# Autodesk Inventor assembly: ZespolDuzegoKola
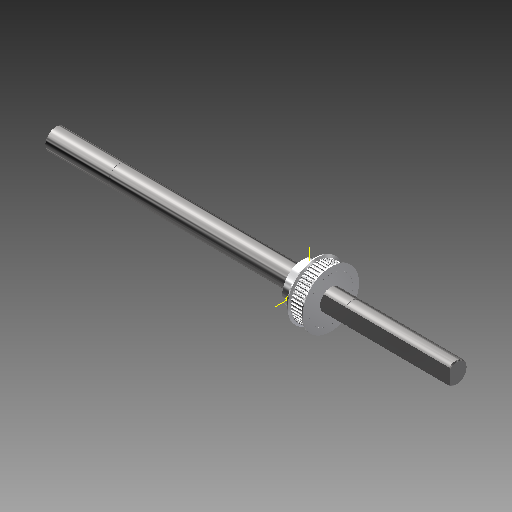
[picture p0: Inventor's stored thumbnail of the model, 512x512]
Saved by Autodesk Inventor 2019 (Build 230136000, 136)
## iProperties
Created: 2020-05-23
Part Number: ZespolDuzegoKola
Document SubType Name: Assembly
Designer: estee
Author: estee
## Documents named in this file (4)
- C:\Users\estee\OneDrive\Pulpit\estere\1\MUM\wogoleNajnowszyGit\Mechanika\Moduł obrotu RET Estera\projejt\projejt\Zlozenie\ModulDuzegoKolaKrotki.iam
- C:\Users\estee\OneDrive\Pulpit\estere\1\MUM\wogoleNajnowszyGit\Mechanika\Moduł obrotu RET Estera\projejt\projejt\Zlozenie\ISO 4029 - M3 x 6 - ISO.ipt
- C:\Users\estee\OneDrive\Pulpit\estere\1\MUM\wogoleNajnowszyGit\Mechanika\Moduł obrotu RET Estera\projejt\projejt\Zlozenie\GT2_50teeth.ipt
- C:\Users\estee\OneDrive\Pulpit\estere\1\MUM\wogoleNajnowszyGit\Mechanika\Moduł obrotu RET Estera\projejt\projejt\Zlozenie\walekREK.ipt
## Components (4 placed, 3 different names)
1. ISO 4029 M3 x 6:1 — Mate:2, Flush:1, Tangent:2
2. ISO 4029 M3 x 6:2 — Mate:3, Tangent:1
3. GT2_50teeth:1 — Mate:1, Mate:2, Mate:3
4. walekREK:1 — Mate:1, Tangent:1, Flush:1, Tangent:2
## Relationships (6: Mate 3, Tangent 2, Flush 1)
- Mate:1: GT2_50teeth:1 ↔ walekREK:1
- Mate:2: ISO 4029 M3 x 6:1 ↔ GT2_50teeth:1
- Mate:3: ISO 4029 M3 x 6:2 ↔ GT2_50teeth:1
- Tangent:1: ISO 4029 M3 x 6:2 ↔ walekREK:1
- Flush:1 (6 mm): ISO 4029 M3 x 6:1 ↔ walekREK:1
- Tangent:2: ISO 4029 M3 x 6:1 ↔ walekREK:1
